# Autodesk Inventor assembly: DriveTrain
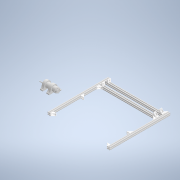
[picture p0: Inventor's stored thumbnail of the model, 180x180]
Saved by Autodesk Inventor 2020.2 (Build 242310000, 310)
## iProperties
Created: 2020-01-29
Part Number: DriveTrain
Document SubType Name: Assembly
Designer: yukin
Author: yukin
## Documents named in this file (7)
- C:\Autodesk\Files\CAD\Robotics 2019-2020\DriveTrain\DriveTrain.iam
- C:\Autodesk\Files\CAD\Robotics 2019-2020\DriveTrain\RevHexMotor\RevHexMotor.iam
- C:\Autodesk\Files\CAD\Robotics 2019-2020\DriveTrain\MotorMount_vCAD.ipt
- C:\Autodesk\Files\CAD\Robotics 2019-2020\DriveTrain\Extrusions\17in.ipt
- C:\Autodesk\Files\CAD\Robotics 2019-2020\DriveTrain\CornerBracket.ipt
- C:\Autodesk\Files\CAD\Robotics 2019-2020\DriveTrain\MotorMountBackSide.ipt
- C:\Autodesk\Files\CAD\Robotics 2019-2020\DriveTrain\Extrusions\18in.ipt
## Components (19 placed, 6 different names)
1. RevHexMotor:1 [sub-assembly] — Rotational:1, Insert:1
2. MotorMount_vCAD:1 — Rotational:1, Flush:21
3. 17in:1 — Mate:1, Flush:1, Flush:2, Flush:12, Flush:13, Mate:7, Mate:8, Flush:14, Flush:15, Mate:11, Flush:19
4. 17in:2 — Flush:3, Mate:2, Flush:4, Flush:8, Flush:9, Mate:5, Flush:10, Mate:6, Flush:11, Mate:12, Flush:28
5. CornerBracket:1 — Flush:3, Mate:2, Flush:4, Flush:24, Mate:14
6. CornerBracket:2 — Mate:1, Flush:1, Flush:2, Flush:22, Flush:23, Mate:13
7. CornerBracket:3 — Mate:8, Flush:14, Flush:15
8. CornerBracket:4 — Flush:12, Flush:13, Mate:7
9. CornerBracket:5 — Flush:8, Flush:9, Mate:5
10. CornerBracket:6 — Flush:10, Mate:6, Flush:11
11. CornerBracket:7 — Mate:11, Flush:19, Flush:25, Mate:15, Flush:26
12. CornerBracket:8 — Mate:12, Flush:27, Mate:16, Flush:28
13. MotorMountBackSide:1 — Insert:1, Flush:21
14. 18in:1 — Flush:25, Mate:15, Flush:26, Flush:27, Mate:16, Flush:29, Flush:30, Mate:17, Flush:31, Mate:18
15. 18in:2 — Flush:22, Flush:23, Mate:13, Flush:24, Mate:14, Flush:32, Mate:19, Flush:33, Mate:20, Flush:34
16. CornerBracket:9 — Flush:32, Mate:19, Flush:33
17. CornerBracket:10 — Mate:20, Flush:34
18. CornerBracket:11 — Flush:29, Flush:30, Mate:17
19. CornerBracket:12 — Flush:31, Mate:18
## Relationships (45: Flush 27, Mate 16, RevoluteJoint 1, Insert 1)
- Rotational:1 [RevoluteJoint]: RevHexMotor:1 ↔ MotorMount_vCAD:1
- Mate:1: 17in:1 ↔ CornerBracket:2
- Flush:1: 17in:1 ↔ CornerBracket:2
- Flush:2: 17in:1 ↔ CornerBracket:2
- Flush:3: 17in:2 ↔ CornerBracket:1
- Mate:2: 17in:2 ↔ CornerBracket:1
- Flush:4: 17in:2 ↔ CornerBracket:1
- Flush:8: 17in:2 ↔ CornerBracket:5
- Flush:9: 17in:2 ↔ CornerBracket:5
- Mate:5: 17in:2 ↔ CornerBracket:5
- Flush:10: 17in:2 ↔ CornerBracket:6
- Mate:6: 17in:2 ↔ CornerBracket:6
- Flush:11: 17in:2 ↔ CornerBracket:6
- Flush:12: 17in:1 ↔ CornerBracket:4
- Flush:13: 17in:1 ↔ CornerBracket:4
- Mate:7: 17in:1 ↔ CornerBracket:4
- Mate:8: 17in:1 ↔ CornerBracket:3
- Flush:14: 17in:1 ↔ CornerBracket:3
- Flush:15: 17in:1 ↔ CornerBracket:3
- Mate:11: 17in:1 ↔ CornerBracket:7
- Flush:19: 17in:1 ↔ CornerBracket:7
- Mate:12: 17in:2 ↔ CornerBracket:8
- Insert:1: RevHexMotor:1 ↔ MotorMountBackSide:1
- Flush:21: MotorMount_vCAD:1 ↔ MotorMountBackSide:1
- Flush:22: CornerBracket:2 ↔ 18in:2
- Flush:23: CornerBracket:2 ↔ 18in:2
- Mate:13: CornerBracket:2 ↔ 18in:2
- Flush:24: CornerBracket:1 ↔ 18in:2
- Mate:14: CornerBracket:1 ↔ 18in:2
- Flush:25: CornerBracket:7 ↔ 18in:1
- Mate:15: CornerBracket:7 ↔ 18in:1
- Flush:26: CornerBracket:7 ↔ 18in:1
- Flush:27: CornerBracket:8 ↔ 18in:1
- Mate:16: CornerBracket:8 ↔ 18in:1
- Flush:28: 17in:2 ↔ CornerBracket:8
- Flush:29: 18in:1 ↔ CornerBracket:11
- Flush:30: 18in:1 ↔ CornerBracket:11
- Mate:17: 18in:1 ↔ CornerBracket:11
- Flush:31: 18in:1 ↔ CornerBracket:12
- Mate:18: 18in:1 ↔ CornerBracket:12
- Flush:32: 18in:2 ↔ CornerBracket:9
- Mate:19: 18in:2 ↔ CornerBracket:9
- Flush:33: 18in:2 ↔ CornerBracket:9
- Mate:20: 18in:2 ↔ CornerBracket:10
- Flush:34: 18in:2 ↔ CornerBracket:10
